# Autodesk Inventor assembly: Assembly2
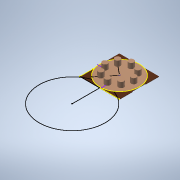
[picture p0: Inventor's stored thumbnail of the model, 180x180]
Saved by Autodesk Inventor 2021.1 (Build 251245010, 245A)
## iProperties
Created: 2024-03-19
Part Number: Assembly2
Document SubType Name: Assembly
Designer: dell
Author: dell
## Documents named in this file (4)
- D:\Projects\Mechatronics system desigen\stp feeding\Assembly2.iam
- D:\Projects\Mechatronics system desigen\stp feeding\feeding_rotating_plate.ipt
- D:\Projects\Mechatronics system desigen\stp feeding\feeding_parts_stand.ipt
- D:\Projects\Mechatronics system desigen\stp feeding\feeding_coupler_Nema17.ipt
## Components (3 placed, 3 different names)
1. feeding_rotating_plate:1 — Mate:1, Mate:2, Mate:3, Mate:4
2. feeding_parts_stand:1 — Mate:5, Mate:6
3. feeding_coupler_Nema17:1 — Mate:1, Mate:2, Mate:3, Mate:4, Mate:5, Mate:6
## Relationships (6: Mate 6)
- Mate:1: feeding_rotating_plate:1 ↔ feeding_coupler_Nema17:1
- Mate:2: feeding_rotating_plate:1 ↔ feeding_coupler_Nema17:1
- Mate:3: feeding_rotating_plate:1 ↔ feeding_coupler_Nema17:1
- Mate:4: feeding_rotating_plate:1 ↔ feeding_coupler_Nema17:1
- Mate:5: feeding_parts_stand:1 ↔ feeding_coupler_Nema17:1
- Mate:6: feeding_parts_stand:1 ↔ feeding_coupler_Nema17:1
